# Autodesk Inventor assembly: Y reduction Assy
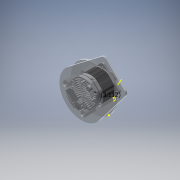
[picture p0: Inventor's stored thumbnail of the model, 180x180]
Saved by Autodesk Inventor 2019 (Build 230136000, 136)
## iProperties
Created: 2018-08-04
Part Number: Y reduction Assy
Document SubType Name: Assembly
Designer: torba
Author: torba
## Documents named in this file (15)
- C:\Users\torba\OneDrive\Documents\Inventor\Plasma 5x10\Y reduction Assy.iam
- C:\Users\torba\OneDrive\Documents\Inventor\Plasma 5x10\CPM-341x\CPM-_ _ _ _ - 3411_-LS.ipt
- C:\Users\torba\OneDrive\Documents\Inventor\Plasma 5x10\PSC1024 Gear (Simplified).ipt
- C:\Users\torba\OneDrive\Documents\Inventor\Plasma 5x10\PARTserver02018080405093218712503063ca5d5\AIS2018\ATP16XL050-A-PUF.iam
- C:\Users\torba\OneDrive\Documents\Inventor\Plasma 5x10\PARTserver02018080405260113312514063ca5d5\AIS2018\ATP50XL050-A-PUF.iam
- C:\Users\torba\OneDrive\Documents\Inventor\Plasma 5x10\AST_Bearings_FR8-2RS\AST_Bearings_FR8-2RS.ipt
- C:\Users\torba\OneDrive\Documents\Inventor\Plasma 5x10\idler.ipt
- C:\Users\torba\OneDrive\Documents\Inventor\Plasma 5x10\y gearing adapter.ipt
- C:\Users\torba\OneDrive\Documents\Inventor\Plasma 5x10\Servo Flange v2.ipt
- C:\Users\torba\OneDrive\Documents\Inventor\Plasma 5x10\belt x.ipt
- C:\Users\torba\OneDrive\Documents\Inventor\Plasma 5x10\keyed shaft 80mm.ipt
- C:\Users\torba\OneDrive\Documents\Inventor\Plasma 5x10\y shaft spacer.ipt
- C:\Users\torba\OneDrive\Documents\Inventor\Plasma 5x10\idler spacer.ipt
- C:\Users\torba\OneDrive\Documents\Inventor\Plasma 5x10\shaft washer 1mm.ipt
- C:\Users\torba\OneDrive\Documents\Inventor\Plasma 5x10\y reduction spacer.ipt
## Components (18 placed, 14 different names)
1. CPM-_ _ _ _ - 3411_-LS:1 — Mate:1, Mate:2, Mate:8, Mate:10, Mate:13, Mate:20
2. Servo Flange v2:1 — Mate:16, Mate:17, Flush:4, Mate:18, Mate:34, Mate:35, Mate:36, Mate:37
3. PSC1024 Gear (Simplified):1 — Mate:5, Mate:7, Mate:9, Flush:4, Mate:21, Mate:23
4. ATP16XL050-A-PUF:1 [sub-assembly] — Flush:1, Mate:1, Mate:19
5. ATP50XL050-A-PUF:1 [sub-assembly] — Flush:1, Mate:2, Flush:2, Mate:5, Mate:6, Mate:12, Mate:14
6. AST_Bearings_FR8-2RS:1 — Mate:7, Mate:11, Mate:12, Mate:22, Mate:28
7. AST_Bearings_FR8-2RS:2 — Mate:6, Mate:14, Mate:16, Mate:17, Mate:24
8. idler:1 — Flush:2, Mate:25, Mate:27
9. y gearing adapter:1 — Mate:8, Mate:9, Mate:10, Mate:11, Mate:13, Mate:18, Flush:5, Mate:26, Mate:27, Mate:30, Mate:31, Mate:32, Mate:33
10. belt x:1 — Mate:19, Mate:20, Mate:21
11. keyed shaft 80mm:1 — Mate:22, Flush:5, Mate:29
12. y shaft spacer:1 — Mate:23, Mate:24
13. idler spacer:1 — Mate:25, Mate:26
14. shaft washer 1mm:1 — Mate:28, Mate:29
15. y reduction spacer:1 — Mate:33, Mate:37
16. y reduction spacer:2 — Mate:32, Mate:36
17. y reduction spacer:3 — Mate:31, Mate:35
18. y reduction spacer:4 — Mate:30, Mate:34
## Relationships (38: Mate 34, Flush 4)
- Flush:1: ATP16XL050-A-PUF:1 ↔ ATP50XL050-A-PUF:1
- Mate:1: CPM-_ _ _ _ - 3411_-LS:1 ↔ ATP16XL050-A-PUF:1
- Mate:2 (110 mm): CPM-_ _ _ _ - 3411_-LS:1 ↔ ATP50XL050-A-PUF:1
- Flush:2 (2.5 mm): ATP50XL050-A-PUF:1 ↔ idler:1
- Mate:5: PSC1024 Gear (Simplified):1 ↔ ATP50XL050-A-PUF:1
- Mate:6: ATP50XL050-A-PUF:1 ↔ AST_Bearings_FR8-2RS:2
- Mate:7: PSC1024 Gear (Simplified):1 ↔ AST_Bearings_FR8-2RS:1
- Mate:8: CPM-_ _ _ _ - 3411_-LS:1 ↔ y gearing adapter:1
- Mate:9: PSC1024 Gear (Simplified):1 ↔ y gearing adapter:1
- Mate:10: CPM-_ _ _ _ - 3411_-LS:1 ↔ y gearing adapter:1
- Mate:11: AST_Bearings_FR8-2RS:1 ↔ y gearing adapter:1
- Mate:12 (1 mm): ATP50XL050-A-PUF:1 ↔ AST_Bearings_FR8-2RS:1
- Mate:13: CPM-_ _ _ _ - 3411_-LS:1 ↔ y gearing adapter:1
- Mate:14 (10 mm): ATP50XL050-A-PUF:1 ↔ AST_Bearings_FR8-2RS:2
- Mate:16: Servo Flange v2:1 ↔ AST_Bearings_FR8-2RS:2
- Mate:17: Servo Flange v2:1 ↔ AST_Bearings_FR8-2RS:2
- Flush:4 (27.7 mm): Servo Flange v2:1 ↔ PSC1024 Gear (Simplified):1
- Mate:18: Servo Flange v2:1 ↔ y gearing adapter:1
- Mate:19 (2 mm): ATP16XL050-A-PUF:1 ↔ belt x:1
- Mate:20: CPM-_ _ _ _ - 3411_-LS:1 ↔ belt x:1
- Mate:21: PSC1024 Gear (Simplified):1 ↔ belt x:1
- Mate:22: AST_Bearings_FR8-2RS:1 ↔ keyed shaft 80mm:1
- Flush:5 (5 mm): y gearing adapter:1 ↔ keyed shaft 80mm:1
- Mate:23: PSC1024 Gear (Simplified):1 ↔ y shaft spacer:1
- Mate:24: AST_Bearings_FR8-2RS:2 ↔ y shaft spacer:1
- Mate:25: idler:1 ↔ idler spacer:1
- Mate:26: y gearing adapter:1 ↔ idler spacer:1
- Mate:27: idler:1 ↔ y gearing adapter:1
- Mate:28: AST_Bearings_FR8-2RS:1 ↔ shaft washer 1mm:1
- Mate:29: keyed shaft 80mm:1 ↔ shaft washer 1mm:1
- Mate:30: y gearing adapter:1 ↔ y reduction spacer:4
- Mate:31: y gearing adapter:1 ↔ y reduction spacer:3
- Mate:32: y gearing adapter:1 ↔ y reduction spacer:2
- Mate:33: y gearing adapter:1 ↔ y reduction spacer:1
- Mate:34: Servo Flange v2:1 ↔ y reduction spacer:4
- Mate:35: Servo Flange v2:1 ↔ y reduction spacer:3
- Mate:36: Servo Flange v2:1 ↔ y reduction spacer:2
- Mate:37: Servo Flange v2:1 ↔ y reduction spacer:1
